# Autodesk Inventor assembly: 100-10-FRAME-CHASSIS-ASM-01
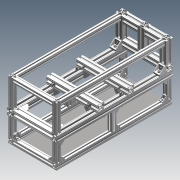
[picture p0: Inventor's stored thumbnail of the model, 180x180]
Saved by Autodesk Inventor 2018.2 (Build 222227000, 227)
## iProperties
Manager: feesmrt
Company: FRANC0R
Created: 2017-12-16
Part Number: 100-10-FRAME-CHASSIS-ASM-01
Material: Generisch
Document SubType Name: Assembly
Designer: feesmrt
Project: Rescue Robot
Cost Center: -
Description: Baseframe ASM
Engineer: feesmrt
Authority: feesmrt
Stock Number: 100-10-FRAME-CHASSIS-ASM-01
Author: feesmrt
Title: Baseframe ASM
Subject: Rescue Robot
Revision Number: 1
## Documents named in this file (16)
- D:\Programmierung\FRANC0R\CAD\02-Rocker-Bogie-Robot\100-CHASSIS\10-FRAME\100-10-FRAME-CHASSIS-ASM-01.iam
- D:\Programmierung\FRANC0R\CAD\02-Rocker-Bogie-Robot\100-CHASSIS\10-FRAME\100-10-FRAME-PROFILE-LENGTH-01.ipt
- D:\Programmierung\FRANC0R\CAD\02-Rocker-Bogie-Robot\100-CHASSIS\10-FRAME\100-10-FRAME-PROFILE-WIDTH-01.ipt
- D:\Programmierung\FRANC0R\CAD\02-Rocker-Bogie-Robot\100-CHASSIS\10-FRAME\100-10-FRAME-PROFILE-WIDTH-02.ipt
- D:\Programmierung\FRANC0R\CAD\02-Rocker-Bogie-Robot\100-CHASSIS\10-FRAME\100-10-FRAME-PROFILE-ROCKER-CONNECTOR.ipt
- D:\Programmierung\FRANC0R\CAD\02-Rocker-Bogie-Robot\900-COMPONENTS\900-50-PROFILES\900-50-PROFILES-ANGLE-CONN-30x30-02.iam
- D:\Programmierung\FRANC0R\CAD\02-Rocker-Bogie-Robot\900-COMPONENTS\900-50-PROFILES\900-50-PROFILES-ANGLE-CONN-30x30-01.iam
- D:\Programmierung\FRANC0R\CAD\02-Rocker-Bogie-Robot\100-CHASSIS\10-FRAME\100-10-FRAME-ROCKER-SCREW-01.iam
- D:\Programmierung\FRANC0R\CAD\02-Rocker-Bogie-Robot\100-CHASSIS\10-FRAME\100-10-FRAME-PROFILE-BOT-H-01.iam
- D:\Programmierung\FRANC0R\CAD\02-Rocker-Bogie-Robot\100-CHASSIS\10-FRAME\100-10-FRAME-PROFILE-BOT-L-01.ipt
- D:\Programmierung\FRANC0R\CAD\02-Rocker-Bogie-Robot\100-CHASSIS\10-FRAME\100-10-FRAME-PROFILE-BOT-W-01.ipt
- D:\Programmierung\FRANC0R\CAD\02-Rocker-Bogie-Robot\900-COMPONENTS\900-50-PROFILES\900-50-PROFILES-ANGLE-CONN-20x20-01.iam
- D:\Programmierung\FRANC0R\CAD\02-Rocker-Bogie-Robot\100-CHASSIS\10-FRAME\100-10-FRAME-BOTTOM-PLATE.iam
- D:\Programmierung\FRANC0R\CAD\02-Rocker-Bogie-Robot\100-CHASSIS\10-FRAME\100-10-FRAME-DIFFERENTIAL-01.iam
- D:\Programmierung\FRANC0R\CAD\02-Rocker-Bogie-Robot\100-CHASSIS\10-FRAME\100-10-FRAME-TOP-01.iam
- D:\Programmierung\FRANC0R\CAD\02-Rocker-Bogie-Robot\100-CHASSIS\Chassis-Dimensions.xlsx
## Components (36 placed, 14 different names)
1. 100-10-FRAME-PROFILE-LENGTH-01:1 — Passend:1, Passend:4, Passend:6, Passend:23, Passend:27, Passend:34, Passend:47, Passend:48, Passend:49, Passend:50, Passend:55, Passend:61, Passend:62, Passend:63, Passend:64, Fluchtend:4, Passend:65, Passend:66, Passend:67, Passend:68, Fluchtend:6
2. 100-10-FRAME-PROFILE-LENGTH-01:2 — Passend:2, Passend:3, Passend:5, Passend:25, Passend:29, Passend:31, Passend:43, Passend:44, Passend:45, Passend:46, Passend:56, Passend:58, Passend:59, Passend:69, Passend:70, Fluchtend:7, Passend:71, Passend:72, Passend:73, Passend:74, Fluchtend:9, Passend:94, Fluchtend:18
3. 100-10-FRAME-PROFILE-WIDTH-01:2 — Passend:10, Passend:11, Passend:12, Passend:32, Passend:33
4. 100-10-FRAME-PROFILE-WIDTH-02:1 — Passend:13, Passend:14, Fluchtend:1, Passend:57, Passend:60, Passend:93, Fluchtend:16, Fluchtend:17
5. 100-10-FRAME-PROFILE-ROCKER-CONNECTOR:1 — Passend:15, Passend:17, Fluchtend:3, Passend:24, Passend:26, Passend:39, Passend:40, Passend:41, Passend:42, Passend:51, Passend:53
6. 100-10-FRAME-PROFILE-ROCKER-CONNECTOR:2 — Passend:16, Passend:18, Fluchtend:2, Passend:28, Passend:30, Passend:35, Passend:36, Passend:37, Passend:38, Passend:52, Passend:54
7. 900-50-PROFILES-ANGLE-CONN-30x30-02:3 [sub-assembly] — Passend:23, Passend:24, Passend:53
8. 900-50-PROFILES-ANGLE-CONN-30x30-02:4 [sub-assembly] — Passend:25, Passend:26, Passend:51
9. 900-50-PROFILES-ANGLE-CONN-30x30-02:5 [sub-assembly] — Passend:27, Passend:28, Passend:54
10. 900-50-PROFILES-ANGLE-CONN-30x30-02:6 [sub-assembly] — Passend:29, Passend:30, Passend:52
11. 900-50-PROFILES-ANGLE-CONN-30x30-01:1 [sub-assembly] — Passend:31, Passend:32, Passend:56
12. 900-50-PROFILES-ANGLE-CONN-30x30-01:2 [sub-assembly] — Passend:33, Passend:34, Passend:55
13. 100-10-FRAME-ROCKER-SCREW-01:1 [sub-assembly] — Passend:35, Passend:36
14. 100-10-FRAME-ROCKER-SCREW-01:2 [sub-assembly] — Passend:37, Passend:38
15. 100-10-FRAME-ROCKER-SCREW-01:3 [sub-assembly] — Passend:39, Passend:40
16. 100-10-FRAME-ROCKER-SCREW-01:4 [sub-assembly] — Passend:41, Passend:42
17. 100-10-FRAME-ROCKER-SCREW-01:5 [sub-assembly] — Passend:43, Passend:44
18. 100-10-FRAME-ROCKER-SCREW-01:6 [sub-assembly] — Passend:49, Passend:50
19. 100-10-FRAME-ROCKER-SCREW-01:7 [sub-assembly] — Passend:47, Passend:48
20. 100-10-FRAME-ROCKER-SCREW-01:8 [sub-assembly] — Passend:45, Passend:46
21. 900-50-PROFILES-ANGLE-CONN-30x30-02:7 [sub-assembly] — Passend:57, Passend:58, Passend:59
22. 900-50-PROFILES-ANGLE-CONN-30x30-02:8 [sub-assembly] — Passend:60, Passend:61, Passend:62
23. 100-10-FRAME-PROFILE-BOT-H-01:1 [sub-assembly] — Passend:63, Passend:64, Fluchtend:4, Passend:75, Fluchtend:10, Passend:76, Passend:91, Passend:92
24. 100-10-FRAME-PROFILE-BOT-H-01:2 [sub-assembly] — Passend:65, Passend:66, Fluchtend:5
25. 100-10-FRAME-PROFILE-BOT-H-01:3 [sub-assembly] — Passend:67, Passend:68, Fluchtend:6
26. 100-10-FRAME-PROFILE-BOT-H-01:4 [sub-assembly] — Passend:69, Passend:70, Fluchtend:7, Passend:77, Fluchtend:11, Passend:78, Passend:87, Passend:89
27. 100-10-FRAME-PROFILE-BOT-H-01:5 [sub-assembly] — Passend:71, Passend:72, Fluchtend:8
28. 100-10-FRAME-PROFILE-BOT-H-01:6 [sub-assembly] — Passend:73, Passend:74, Fluchtend:9
29. 100-10-FRAME-PROFILE-BOT-L-01:1 — Passend:75, Fluchtend:10, Passend:76, Passend:79, Fluchtend:12, Fluchtend:13, Passend:86, Fluchtend:14
30. 100-10-FRAME-PROFILE-BOT-L-01:2 — Passend:77, Fluchtend:11, Passend:78
31. 100-10-FRAME-PROFILE-BOT-W-01:1 — Passend:79, Fluchtend:12, Fluchtend:13, Fluchtend:15, Passend:88, Passend:90
32. 900-50-PROFILES-ANGLE-CONN-20x20-01:1 [sub-assembly] — Passend:90, Passend:91, Passend:92
33. 900-50-PROFILES-ANGLE-CONN-20x20-01:2 [sub-assembly] — Passend:87, Passend:88, Passend:89
34. 100-10-FRAME-BOTTOM-PLATE:1 [sub-assembly] — Passend:86, Fluchtend:14, Fluchtend:15
35. 100-10-FRAME-DIFFERENTIAL-01:1 [sub-assembly] — Passend:93, Fluchtend:16, Fluchtend:17
36. 100-10-FRAME-TOP-01:1 [sub-assembly] — Passend:94, Passend:95, Fluchtend:18
## Relationships (100: Mate 82, Flush 18)
- Passend:1 [Mate]: 100-10-FRAME-PROFILE-LENGTH-01:1
- Passend:2 [Mate]: 100-10-FRAME-PROFILE-LENGTH-01:2
- Passend:3 [Mate]: 100-10-FRAME-PROFILE-LENGTH-01:2
- Passend:4 [Mate]: 100-10-FRAME-PROFILE-LENGTH-01:1
- Passend:5 [Mate] (-95 mm): 100-10-FRAME-PROFILE-LENGTH-01:2
- Passend:6 [Mate] (95 mm): 100-10-FRAME-PROFILE-LENGTH-01:1
- Passend:10 [Mate]: 100-10-FRAME-PROFILE-WIDTH-01:2
- Passend:11 [Mate]: 100-10-FRAME-PROFILE-WIDTH-01:2
- Passend:12 [Mate] (-235 mm): 100-10-FRAME-PROFILE-WIDTH-01:2
- Passend:13 [Mate] (30 mm): 100-10-FRAME-PROFILE-WIDTH-02:1
- Passend:14 [Mate]: 100-10-FRAME-PROFILE-WIDTH-02:1
- Fluchtend:1 [Flush] (235 mm): 100-10-FRAME-PROFILE-WIDTH-02:1
- Passend:15 [Mate] (30 mm): 100-10-FRAME-PROFILE-ROCKER-CONNECTOR:1
- Passend:16 [Mate] (30 mm): 100-10-FRAME-PROFILE-ROCKER-CONNECTOR:2
- Passend:17 [Mate]: 100-10-FRAME-PROFILE-ROCKER-CONNECTOR:1
- Passend:18 [Mate]: 100-10-FRAME-PROFILE-ROCKER-CONNECTOR:2
- Fluchtend:2 [Flush] (65 mm): 100-10-FRAME-PROFILE-ROCKER-CONNECTOR:2
- Fluchtend:3 [Flush] (-65 mm): 100-10-FRAME-PROFILE-ROCKER-CONNECTOR:1
- Passend:23 [Mate]: 100-10-FRAME-PROFILE-LENGTH-01:1 ↔ 900-50-PROFILES-ANGLE-CONN-30x30-02:3
- Passend:24 [Mate]: 100-10-FRAME-PROFILE-ROCKER-CONNECTOR:1 ↔ 900-50-PROFILES-ANGLE-CONN-30x30-02:3
- Passend:25 [Mate]: 100-10-FRAME-PROFILE-LENGTH-01:2 ↔ 900-50-PROFILES-ANGLE-CONN-30x30-02:4
- Passend:26 [Mate]: 100-10-FRAME-PROFILE-ROCKER-CONNECTOR:1 ↔ 900-50-PROFILES-ANGLE-CONN-30x30-02:4
- Passend:27 [Mate]: 100-10-FRAME-PROFILE-LENGTH-01:1 ↔ 900-50-PROFILES-ANGLE-CONN-30x30-02:5
- Passend:28 [Mate]: 100-10-FRAME-PROFILE-ROCKER-CONNECTOR:2 ↔ 900-50-PROFILES-ANGLE-CONN-30x30-02:5
- Passend:29 [Mate]: 100-10-FRAME-PROFILE-LENGTH-01:2 ↔ 900-50-PROFILES-ANGLE-CONN-30x30-02:6
- Passend:30 [Mate]: 100-10-FRAME-PROFILE-ROCKER-CONNECTOR:2 ↔ 900-50-PROFILES-ANGLE-CONN-30x30-02:6
- Passend:31 [Mate]: 100-10-FRAME-PROFILE-LENGTH-01:2 ↔ 900-50-PROFILES-ANGLE-CONN-30x30-01:1
- Passend:32 [Mate]: 100-10-FRAME-PROFILE-WIDTH-01:2 ↔ 900-50-PROFILES-ANGLE-CONN-30x30-01:1
- Passend:33 [Mate]: 100-10-FRAME-PROFILE-WIDTH-01:2 ↔ 900-50-PROFILES-ANGLE-CONN-30x30-01:2
- Passend:34 [Mate]: 100-10-FRAME-PROFILE-LENGTH-01:1 ↔ 900-50-PROFILES-ANGLE-CONN-30x30-01:2
- Passend:35 [Mate]: 100-10-FRAME-PROFILE-ROCKER-CONNECTOR:2 ↔ 100-10-FRAME-ROCKER-SCREW-01:1
- Passend:36 [Mate]: 100-10-FRAME-PROFILE-ROCKER-CONNECTOR:2 ↔ 100-10-FRAME-ROCKER-SCREW-01:1
- Passend:37 [Mate]: 100-10-FRAME-PROFILE-ROCKER-CONNECTOR:2 ↔ 100-10-FRAME-ROCKER-SCREW-01:2
- Passend:38 [Mate]: 100-10-FRAME-PROFILE-ROCKER-CONNECTOR:2 ↔ 100-10-FRAME-ROCKER-SCREW-01:2
- Passend:39 [Mate]: 100-10-FRAME-PROFILE-ROCKER-CONNECTOR:1 ↔ 100-10-FRAME-ROCKER-SCREW-01:3
- Passend:40 [Mate]: 100-10-FRAME-PROFILE-ROCKER-CONNECTOR:1 ↔ 100-10-FRAME-ROCKER-SCREW-01:3
- Passend:41 [Mate]: 100-10-FRAME-PROFILE-ROCKER-CONNECTOR:1 ↔ 100-10-FRAME-ROCKER-SCREW-01:4
- Passend:42 [Mate]: 100-10-FRAME-PROFILE-ROCKER-CONNECTOR:1 ↔ 100-10-FRAME-ROCKER-SCREW-01:4
- Passend:43 [Mate]: 100-10-FRAME-PROFILE-LENGTH-01:2 ↔ 100-10-FRAME-ROCKER-SCREW-01:5
- Passend:44 [Mate]: 100-10-FRAME-PROFILE-LENGTH-01:2 ↔ 100-10-FRAME-ROCKER-SCREW-01:5
- Passend:45 [Mate]: 100-10-FRAME-PROFILE-LENGTH-01:2 ↔ 100-10-FRAME-ROCKER-SCREW-01:8
- Passend:46 [Mate]: 100-10-FRAME-PROFILE-LENGTH-01:2 ↔ 100-10-FRAME-ROCKER-SCREW-01:8
- Passend:47 [Mate]: 100-10-FRAME-PROFILE-LENGTH-01:1 ↔ 100-10-FRAME-ROCKER-SCREW-01:7
- Passend:48 [Mate]: 100-10-FRAME-PROFILE-LENGTH-01:1 ↔ 100-10-FRAME-ROCKER-SCREW-01:7
- Passend:49 [Mate]: 100-10-FRAME-PROFILE-LENGTH-01:1 ↔ 100-10-FRAME-ROCKER-SCREW-01:6
- Passend:50 [Mate]: 100-10-FRAME-PROFILE-LENGTH-01:1 ↔ 100-10-FRAME-ROCKER-SCREW-01:6
- Passend:51 [Mate]: 100-10-FRAME-PROFILE-ROCKER-CONNECTOR:1 ↔ 900-50-PROFILES-ANGLE-CONN-30x30-02:4
- Passend:52 [Mate]: 100-10-FRAME-PROFILE-ROCKER-CONNECTOR:2 ↔ 900-50-PROFILES-ANGLE-CONN-30x30-02:6
- Passend:53 [Mate]: 100-10-FRAME-PROFILE-ROCKER-CONNECTOR:1 ↔ 900-50-PROFILES-ANGLE-CONN-30x30-02:3
- Passend:54 [Mate]: 100-10-FRAME-PROFILE-ROCKER-CONNECTOR:2 ↔ 900-50-PROFILES-ANGLE-CONN-30x30-02:5
- Passend:55 [Mate]: 100-10-FRAME-PROFILE-LENGTH-01:1 ↔ 900-50-PROFILES-ANGLE-CONN-30x30-01:2
- Passend:56 [Mate]: 100-10-FRAME-PROFILE-LENGTH-01:2 ↔ 900-50-PROFILES-ANGLE-CONN-30x30-01:1
- Passend:57 [Mate]: 100-10-FRAME-PROFILE-WIDTH-02:1 ↔ 900-50-PROFILES-ANGLE-CONN-30x30-02:7
- Passend:58 [Mate]: 100-10-FRAME-PROFILE-LENGTH-01:2 ↔ 900-50-PROFILES-ANGLE-CONN-30x30-02:7
- Passend:59 [Mate]: 100-10-FRAME-PROFILE-LENGTH-01:2 ↔ 900-50-PROFILES-ANGLE-CONN-30x30-02:7
- Passend:60 [Mate]: 100-10-FRAME-PROFILE-WIDTH-02:1 ↔ 900-50-PROFILES-ANGLE-CONN-30x30-02:8
- Passend:61 [Mate]: 100-10-FRAME-PROFILE-LENGTH-01:1 ↔ 900-50-PROFILES-ANGLE-CONN-30x30-02:8
- Passend:62 [Mate]: 100-10-FRAME-PROFILE-LENGTH-01:1 ↔ 900-50-PROFILES-ANGLE-CONN-30x30-02:8
- Passend:63 [Mate]: 100-10-FRAME-PROFILE-LENGTH-01:1 ↔ 100-10-FRAME-PROFILE-BOT-H-01:1
- Passend:64 [Mate]: 100-10-FRAME-PROFILE-LENGTH-01:1 ↔ 100-10-FRAME-PROFILE-BOT-H-01:1
- Fluchtend:4 [Flush]: 100-10-FRAME-PROFILE-LENGTH-01:1 ↔ 100-10-FRAME-PROFILE-BOT-H-01:1
- Passend:65 [Mate]: 100-10-FRAME-PROFILE-LENGTH-01:1 ↔ 100-10-FRAME-PROFILE-BOT-H-01:2
- Passend:66 [Mate]: 100-10-FRAME-PROFILE-LENGTH-01:1 ↔ 100-10-FRAME-PROFILE-BOT-H-01:2
- Fluchtend:5 [Flush]: 100-10-FRAME-PROFILE-BOT-H-01:2
- Passend:67 [Mate]: 100-10-FRAME-PROFILE-LENGTH-01:1 ↔ 100-10-FRAME-PROFILE-BOT-H-01:3
- Passend:68 [Mate]: 100-10-FRAME-PROFILE-LENGTH-01:1 ↔ 100-10-FRAME-PROFILE-BOT-H-01:3
- Fluchtend:6 [Flush]: 100-10-FRAME-PROFILE-LENGTH-01:1 ↔ 100-10-FRAME-PROFILE-BOT-H-01:3
- Passend:69 [Mate]: 100-10-FRAME-PROFILE-LENGTH-01:2 ↔ 100-10-FRAME-PROFILE-BOT-H-01:4
- Passend:70 [Mate]: 100-10-FRAME-PROFILE-LENGTH-01:2 ↔ 100-10-FRAME-PROFILE-BOT-H-01:4
- Fluchtend:7 [Flush]: 100-10-FRAME-PROFILE-LENGTH-01:2 ↔ 100-10-FRAME-PROFILE-BOT-H-01:4
- Passend:71 [Mate]: 100-10-FRAME-PROFILE-LENGTH-01:2 ↔ 100-10-FRAME-PROFILE-BOT-H-01:5
- Passend:72 [Mate]: 100-10-FRAME-PROFILE-LENGTH-01:2 ↔ 100-10-FRAME-PROFILE-BOT-H-01:5
- Fluchtend:8 [Flush]: 100-10-FRAME-PROFILE-BOT-H-01:5
- Passend:73 [Mate]: 100-10-FRAME-PROFILE-LENGTH-01:2 ↔ 100-10-FRAME-PROFILE-BOT-H-01:6
- Passend:74 [Mate]: 100-10-FRAME-PROFILE-LENGTH-01:2 ↔ 100-10-FRAME-PROFILE-BOT-H-01:6
- Fluchtend:9 [Flush]: 100-10-FRAME-PROFILE-LENGTH-01:2 ↔ 100-10-FRAME-PROFILE-BOT-H-01:6
- Passend:75 [Mate]: 100-10-FRAME-PROFILE-BOT-H-01:1 ↔ 100-10-FRAME-PROFILE-BOT-L-01:1
- Fluchtend:10 [Flush]: 100-10-FRAME-PROFILE-BOT-H-01:1 ↔ 100-10-FRAME-PROFILE-BOT-L-01:1
- Passend:76 [Mate]: 100-10-FRAME-PROFILE-BOT-H-01:1 ↔ 100-10-FRAME-PROFILE-BOT-L-01:1
- Passend:77 [Mate]: 100-10-FRAME-PROFILE-BOT-H-01:4 ↔ 100-10-FRAME-PROFILE-BOT-L-01:2
- Fluchtend:11 [Flush]: 100-10-FRAME-PROFILE-BOT-H-01:4 ↔ 100-10-FRAME-PROFILE-BOT-L-01:2
- Passend:78 [Mate]: 100-10-FRAME-PROFILE-BOT-H-01:4 ↔ 100-10-FRAME-PROFILE-BOT-L-01:2
- Passend:79 [Mate]: 100-10-FRAME-PROFILE-BOT-L-01:1 ↔ 100-10-FRAME-PROFILE-BOT-W-01:1
- Fluchtend:12 [Flush]: 100-10-FRAME-PROFILE-BOT-L-01:1 ↔ 100-10-FRAME-PROFILE-BOT-W-01:1
- Fluchtend:13 [Flush]: 100-10-FRAME-PROFILE-BOT-L-01:1 ↔ 100-10-FRAME-PROFILE-BOT-W-01:1
- Passend:86 [Mate]: 100-10-FRAME-PROFILE-BOT-L-01:1 ↔ 100-10-FRAME-BOTTOM-PLATE:1
- Fluchtend:14 [Flush]: 100-10-FRAME-PROFILE-BOT-L-01:1 ↔ 100-10-FRAME-BOTTOM-PLATE:1
- Fluchtend:15 [Flush]: 100-10-FRAME-PROFILE-BOT-W-01:1 ↔ 100-10-FRAME-BOTTOM-PLATE:1
- Passend:87 [Mate]: 100-10-FRAME-PROFILE-BOT-H-01:4 ↔ 900-50-PROFILES-ANGLE-CONN-20x20-01:2
- Passend:88 [Mate]: 100-10-FRAME-PROFILE-BOT-W-01:1 ↔ 900-50-PROFILES-ANGLE-CONN-20x20-01:2
- Passend:89 [Mate]: 100-10-FRAME-PROFILE-BOT-H-01:4 ↔ 900-50-PROFILES-ANGLE-CONN-20x20-01:2
- Passend:90 [Mate]: 100-10-FRAME-PROFILE-BOT-W-01:1 ↔ 900-50-PROFILES-ANGLE-CONN-20x20-01:1
- Passend:91 [Mate]: 100-10-FRAME-PROFILE-BOT-H-01:1 ↔ 900-50-PROFILES-ANGLE-CONN-20x20-01:1
- Passend:92 [Mate]: 100-10-FRAME-PROFILE-BOT-H-01:1 ↔ 900-50-PROFILES-ANGLE-CONN-20x20-01:1
- Passend:93 [Mate]: 100-10-FRAME-PROFILE-WIDTH-02:1 ↔ 100-10-FRAME-DIFFERENTIAL-01:1
- Fluchtend:16 [Flush]: 100-10-FRAME-PROFILE-WIDTH-02:1 ↔ 100-10-FRAME-DIFFERENTIAL-01:1
- Fluchtend:17 [Flush]: 100-10-FRAME-PROFILE-WIDTH-02:1 ↔ 100-10-FRAME-DIFFERENTIAL-01:1
- Passend:94 [Mate]: 100-10-FRAME-PROFILE-LENGTH-01:2 ↔ 100-10-FRAME-TOP-01:1
- Passend:95 [Mate]: 100-10-FRAME-TOP-01:1
- Fluchtend:18 [Flush]: 100-10-FRAME-PROFILE-LENGTH-01:2 ↔ 100-10-FRAME-TOP-01:1
## Named parameters: Chassis_Length = 500 mm, Chassis_Width = 220 mm, Chassis_Frame_Size = 30 mm, Rocker_Bearing_Size = 100 mm, Rocker_Screw_Distance = 32.5 mm, Rocker_Screw_Distance_Bottom = 76 mm, Chassis_Bottom_Height = 80 mm
